# Autodesk Inventor assembly: Robot
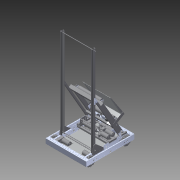
[picture p0: Inventor's stored thumbnail of the model, 180x180]
Saved by Autodesk Inventor 2015 SP1 (Build 190203100, 203)
## iProperties
Created: 2015-01-17
Part Number: Robot
Document SubType Name: Assembly
Designer: Jarod
Author: Jarod
## Documents named in this file (4)
- C:\Users\Jarod\Documents\Westview\Robotics\FRC\2015\CAD\Robot\Robot.iam
- C:\Users\Jarod\Documents\Westview\Robotics\FRC\2015\CAD\Robot\Chassis\Chassis.iam
- C:\Users\Jarod\Documents\Westview\Robotics\FRC\2015\CAD\Robot\Noodle Sucker\Noodle Sucker.iam
- C:\Users\Jarod\Documents\Westview\Robotics\FRC\2015\CAD\Robot\Vertical Lift\Vertical Lift.iam
## Components (3 placed, 3 different names)
1. Chassis:1 [sub-assembly] — Mate:3, Mate:4, Mate:5, Mate:6, Mate:7
2. Noodle Sucker:1 [sub-assembly] — Mate:6, Mate:7
3. Vertical Lift:1 [sub-assembly] — Mate:3, Mate:4, Mate:5
## Relationships (5: Mate 5)
- Mate:3: Chassis:1 ↔ Vertical Lift:1
- Mate:4: Chassis:1 ↔ Vertical Lift:1
- Mate:5: Chassis:1 ↔ Vertical Lift:1
- Mate:6: Chassis:1 ↔ Noodle Sucker:1
- Mate:7: Chassis:1 ↔ Noodle Sucker:1
